# Autodesk Inventor assembly: Wrist
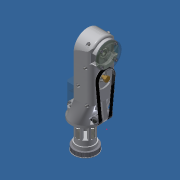
[picture p0: Inventor's stored thumbnail of the model, 180x180]
Saved by Autodesk Inventor 2016 (Build 200138000, 138)
## iProperties
Created: 2015-08-25
Part Number: Wrist
Material: Generisch
Document SubType Name: Assembly
Designer: 4ndreas
Mass: 901.602 g
Surface Area: 1453.73 cm^2
Volume: 401.24 cm^3
Density: 2.24704 g/cm^3
Author: 4ndreas
## Documents named in this file (29)
- C:\Users\4ndreas\Documents\Inventor\RobotARM v2\v4\Wrist.iam
- C:\Users\4ndreas\Documents\Inventor\RobotARM v2\v4\Wrist_A.ipt
- C:\Users\4ndreas\Documents\Inventor\RobotARM v2\v4\Nema17 48.ipt
- C:\Users\4ndreas\Documents\Inventor\RobotARM v2\v4\Wrist\Konstruktions-Assistent\Übertragung des Zahnriemens1.iam
- C:\Users\4ndreas\Documents\Inventor\RobotARM v2\v4\DIN 625 SKF - SKF 624_flansch.ipt
- C:\Users\4ndreas\Documents\Inventor\RobotARM v2\v4\Synchrone Riemenscheibe16.ipt
- C:\Users\4ndreas\Documents\Inventor\Content Center Files\R2014\de-DE\DIN BEARING(1)\DIN 625 SKF - SKF 626.ipt
- C:\Users\4ndreas\Documents\Inventor\Content Center Files\R2014\de-DE\DIN BEARING(1)\DIN 625 SKF - SKF 608.ipt
- C:\Users\4ndreas\Documents\Inventor\Content Center Files\R2014\de-DE\DIN BEARING(1)\DIN 625 SKF - SKF 624.ipt
- C:\Users\4ndreas\Documents\Inventor\Content Center Files\R2014\de-DE\ISO 7380-1\ISO 7380-1 - M4 x 30.ipt
- C:\Users\4ndreas\Documents\Inventor\Content Center Files\R2014\de-DE\ISO 7380-1\ISO 7380-1 - M4 x 35.ipt
- C:\Users\4ndreas\Documents\Inventor\RobotARM v2\v4\Twisted_Belt.ipt
- C:\Users\4ndreas\Documents\Inventor\RobotARM v2\v2\encoder.iam
- C:\Users\4ndreas\Documents\Inventor\Content Center Files\R2014\de-DE\DIN 125-1  A\DIN 125 - A 4,3.ipt
- C:\Users\4ndreas\Documents\Inventor\Content Center Files\R2014\de-DE\DIN 912\DIN 912 - M4 x 0,7 x 20 x 18,25.ipt
- C:\Users\4ndreas\Documents\Inventor\Content Center Files\R2014\de-DE\DIN 934\DIN 934 - M4 x 0,7.ipt
- C:\Users\4ndreas\Documents\Inventor\Content Center Files\R2014\de-DE\DIN 912\DIN 912 - M3 x 0,5 x 16 x 14,75.ipt
- C:\Users\4ndreas\Documents\Inventor\Content Center Files\R2014\de-DE\DIN 125-1  A\DIN 125 - A 3,2.ipt
- C:\Users\4ndreas\Documents\Inventor\Content Center Files\R2014\de-DE\DIN 7991(2)\DIN 7991 - M3x10.ipt
- C:\Users\4ndreas\Documents\Inventor\Content Center Files\R2014\de-DE\DIN 912\DIN 912 - M4 x 0,7 x 40 x 20.ipt
- C:\Users\4ndreas\Documents\Inventor\RobotARM v2\v4\RotoatorGear.ipt
- C:\Users\4ndreas\Documents\Inventor\Content Center Files\R2014\de-DE\DIN 933\DIN 933 - M4  x 30.ipt
- C:\Users\4ndreas\Documents\Inventor\Content Center Files\R2014\de-DE\DIN 912\DIN 912 - M4 x 0,7 x 30 x 20.ipt
- C:\Users\4ndreas\Documents\Inventor\RobotARM v2\v4\T25-06-44_2.ipt
- C:\Users\4ndreas\Documents\Inventor\RobotARM v2\v4\Bolzen6mm.ipt
- C:\Users\4ndreas\Documents\Inventor\RobotARM v2\Diszanzbolzen_M4x20.ipt
- C:\Users\4ndreas\Documents\Inventor\RobotARM v2\v4\DIN 912 - M4 x 0,7 x55.ipt
- C:\Users\4ndreas\Documents\Inventor\Content Center Files\R2014\de-DE\DIN 985\DIN 985 - M4.ipt
- C:\Users\4ndreas\Documents\Inventor\Content Center Files\R2014\de-DE\DIN 562\DIN 562 - M4 x 7.ipt
## Components (68 placed, 28 different names)
1. Wrist_A:1 — Passend:1, Winkel:1, Passend:2, Winkel:2, Fluchtend:1, Fluchtend:2, Passend:5, Passend:8, Passend:11, Passend:12, Passend:14, Passend:15, Fluchtend:4, Passend:20, Passend:22, Passend:23, Passend:24, Passend:34, Passend:39, Passend:40, Winkel:3, Passend:51, Passend:54, Passend:58, Passend:59, Passend:61, Passend:62, Passend:66, Passend:67, Passend:70, Passend:71, Passend:77, Passend:78, Passend:79, Passend:80, Passend:81, Passend:82, Passend:83, Passend:84, Passend:85, Passend:94, Passend:95, Passend:96, Passend:97, Passend:102, Passend:103, Passend:105, Passend:120, Passend:121, Passend:122, Passend:123, Passend:124, Passend:125, Passend:126, Passend:127, Passend:128, Passend:129, Passend:130, Passend:131, Passend:159, Passend:161, Passend:162
2. Nema17 48:1 — Passend:1, Winkel:1, Fluchtend:1, Passend:6, Passend:7, Passend:98, Passend:99, Passend:100, Passend:101
3. Übertragung des Zahnriemens:1 [sub-assembly] — Passend:13, Passend:21, Passend:27, Passend:31, Passend:48
4. F624 ZZ 4x13x5:2 — Passend:3, Passend:4, Passend:35
5. F624 ZZ 4x13x5:3 — Passend:3, Passend:4, Passend:5, Passend:8, Fluchtend:6, Passend:36
6. Synchrone Riemenscheibe1:1 — Passend:6, Passend:7, Fluchtend:5, Fluchtend:8, Passend:38
7. F624 ZZ 4x13x5:4 — Passend:9, Passend:10, Passend:11, Passend:12
8. F624 ZZ 4x13x5:5 — Passend:9, Passend:10, Passend:44
9. Synchrone Riemenscheibe1:2 — Passend:13, Passend:19
10. DIN 625 SKF SKF 626:1 — Passend:14, Fluchtend:4, Passend:154, Passend:157
11. DIN 625 SKF SKF 626:2 — Passend:15, Passend:19, Passend:20
12. DIN 625 SKF SKF 608:1 — Passend:22, Passend:24
13. DIN 625 SKF SKF 608:2 — Passend:21, Passend:23
14. DIN 625 SKF SKF 624:6 — Passend:25, Passend:26, Passend:27, Passend:32
15. DIN 625 SKF SKF 624:7 — Passend:25, Passend:26
16. DIN 125-1 A A 4,3:6
17. ISO 7380-1 M4 x 30:1 — Passend:31, Passend:32, Passend:160
18. ISO 7380-1 M4 x 35:1 — Passend:34, Passend:35, Passend:43
19. Twisted_Belt:1 — Fluchtend:5, Fluchtend:6, Passend:36, Fluchtend:8, Passend:38
20. DIN 985 - ersetzt durch DIN EN ISO 10511 M4:1 — Passend:43, Passend:44
21. encoder:1 [sub-assembly] — Passend:48, Winkel:3, Winkel:4, Passend:104, Passend:159
22. DIN 912 - ersetzt durch DIN EN ISO 4762 M4 x 55:1 — Passend:51, Passend:52, Passend:53, Passend:75
23. DIN 912 - ersetzt durch DIN EN ISO 4762 M4 x 55:2 — Passend:56, Passend:59, Passend:64, Passend:73
24. DIN 912 - ersetzt durch DIN EN ISO 4762 M4 x 55:3 — Passend:57, Passend:58, Passend:65, Passend:74
25. DIN 125-1 A A 4,3:1 — Passend:52, Passend:53, Passend:54
26. DIN 125-1 A A 4,3:2 — Passend:57, Passend:65, Passend:66
27. DIN 125-1 A A 4,3:3 — Passend:56, Passend:64, Passend:67
28. DIN 125-1 A A 4,3:4 — Passend:60, Passend:62, Passend:63
29. DIN 912 - ersetzt durch DIN EN ISO 4762 M4 x 40:5 — Passend:60, Passend:61, Passend:63, Passend:72
30. DIN 912 - ersetzt durch DIN EN ISO 4762 M4 x 20:1 — Passend:68, Passend:69, Passend:71, Passend:76
31. DIN 125-1 A A 4,3:5 — Passend:68, Passend:69, Passend:70
32. DIN 934 - ersetzt durch DIN EN 24032/28673/28674 M4:1 — Passend:72, Passend:79, Passend:85
33. DIN 934 - ersetzt durch DIN EN 24032/28673/28674 M4:2 — Passend:73, Passend:80, Passend:84
34. DIN 934 - ersetzt durch DIN EN 24032/28673/28674 M4:3 — Passend:74, Passend:81, Passend:82
35. DIN 934 - ersetzt durch DIN EN 24032/28673/28674 M4:4 — Passend:75, Passend:83
36. DIN 934 - ersetzt durch DIN EN 24032/28673/28674 M4:5 — Passend:76, Passend:77, Passend:78
37. DIN 912 - ersetzt durch DIN EN ISO 4762 M3 x 16:1 — Passend:89, Passend:90, Passend:101
38. DIN 912 - ersetzt durch DIN EN ISO 4762 M3 x 16:2 — Passend:88, Passend:91, Passend:99
39. DIN 912 - ersetzt durch DIN EN ISO 4762 M3 x 16:3 — Passend:87, Passend:92, Passend:98
40. DIN 912 - ersetzt durch DIN EN ISO 4762 M3 x 16:4 — Passend:86, Passend:93, Passend:100
41. DIN 125-1 A A 3,2:1 — Passend:86, Passend:93, Passend:94
42. DIN 125-1 A A 3,2:2 — Passend:89, Passend:90, Passend:97
43. DIN 125-1 A A 3,2:3 — Passend:88, Passend:91, Passend:96
44. DIN 125-1 A A 3,2:4 — Passend:87, Passend:92, Passend:95
45. DIN 7991 M3x10:1 — Passend:105, Fluchtend:11, Fluchtend:12
46. DIN 7991 M3x10:2 — Passend:103, Fluchtend:10, Fluchtend:11
47. DIN 7991 M3x10:3 — Passend:104, Fluchtend:12
48. DIN 7991 M3x10:4 — Passend:102, Fluchtend:10
49. RotoatorGear:1 — Passend:120, Passend:121, Passend:122, Passend:136, Passend:137, Passend:138, Passend:139, Passend:148, Passend:149
50. DIN 933 - ersetzt durch DIN EN 24017 M4  x 30:4 — Passend:123, Fluchtend:16, Fluchtend:17, Passend:130, Passend:131, Passend:135
51. DIN 933 - ersetzt durch DIN EN 24017 M4  x 30:3 — Passend:124, Fluchtend:17, Passend:129, Passend:134
52. DIN 933 - ersetzt durch DIN EN 24017 M4  x 30:2 — Passend:125, Fluchtend:15, Passend:128, Passend:133
53. DIN 933 - ersetzt durch DIN EN 24017 M4  x 30:1 — Passend:126, Fluchtend:15, Fluchtend:16, Passend:127, Passend:132
54. Diszanzbolzen_M4x20:5 — Passend:132, Passend:138, Passend:152
55. Diszanzbolzen_M4x20:6 — Passend:133, Passend:139, Passend:151
56. Diszanzbolzen_M4x20:7 — Passend:134, Passend:137, Passend:150
57. Diszanzbolzen_M4x20:8 — Passend:135, Passend:136
58. DIN 125-1 A A 4,3:7
59. DIN 125-1 A A 4,3:8
60. DIN 125-1 A A 4,3:9
61. DIN 125-1 A A 4,3:10
62. DIN 912 - ersetzt durch DIN EN ISO 4762 M4 x 30:1 — Fluchtend:20, Passend:150
63. DIN 912 - ersetzt durch DIN EN ISO 4762 M4 x 30:2 — Fluchtend:19, Fluchtend:20, Passend:152
64. DIN 912 - ersetzt durch DIN EN ISO 4762 M4 x 30:3 — Fluchtend:18, Fluchtend:19, Passend:151
65. DIN 912 - ersetzt durch DIN EN ISO 4762 M4 x 30:4 — Passend:148, Passend:149, Fluchtend:18
66. T25-06-44_2:1 — Passend:154, Passend:155, Passend:156, Passend:158
67. Bolzen6mm:1 — Passend:155, Passend:156, Passend:157, Passend:158
68. DIN 562 M4:1 — Passend:160, Passend:161, Passend:162
## Relationships (155: Mate 136, Flush 15, Angle 4)
- Passend:1 [Mate]: Wrist_A:1 ↔ Nema17 48:1
- Winkel:1 [Angle] (0 deg): Wrist_A:1 ↔ Nema17 48:1
- Passend:2 [Mate]: Wrist_A:1
- Winkel:2 [Angle] (90 deg): Wrist_A:1
- Fluchtend:1 [Flush] (20 mm): Wrist_A:1 ↔ Nema17 48:1
- Fluchtend:2 [Flush]: Wrist_A:1
- Passend:3 [Mate]: F624 ZZ 4x13x5:2 ↔ F624 ZZ 4x13x5:3
- Passend:4 [Mate]: F624 ZZ 4x13x5:2 ↔ F624 ZZ 4x13x5:3
- Passend:5 [Mate]: Wrist_A:1 ↔ F624 ZZ 4x13x5:3
- Passend:6 [Mate] (4.5 mm): Nema17 48:1 ↔ Synchrone Riemenscheibe1:1
- Passend:7 [Mate]: Nema17 48:1 ↔ Synchrone Riemenscheibe1:1
- Passend:8 [Mate]: Wrist_A:1 ↔ F624 ZZ 4x13x5:3
- Passend:9 [Mate]: F624 ZZ 4x13x5:4 ↔ F624 ZZ 4x13x5:5
- Passend:10 [Mate]: F624 ZZ 4x13x5:4 ↔ F624 ZZ 4x13x5:5
- Passend:11 [Mate]: Wrist_A:1 ↔ F624 ZZ 4x13x5:4
- Passend:12 [Mate]: Wrist_A:1 ↔ F624 ZZ 4x13x5:4
- Passend:13 [Mate]: Übertragung des Zahnriemens:1 ↔ Synchrone Riemenscheibe1:2
- Passend:14 [Mate]: Wrist_A:1 ↔ DIN 625 SKF SKF 626:1
- Passend:15 [Mate]: Wrist_A:1 ↔ DIN 625 SKF SKF 626:2
- Fluchtend:4 [Flush]: Wrist_A:1 ↔ DIN 625 SKF SKF 626:1
- Passend:19 [Mate]: Synchrone Riemenscheibe1:2 ↔ DIN 625 SKF SKF 626:2
- Passend:20 [Mate]: Wrist_A:1 ↔ DIN 625 SKF SKF 626:2
- Passend:21 [Mate]: Übertragung des Zahnriemens:1 ↔ DIN 625 SKF SKF 608:2
- Passend:22 [Mate]: Wrist_A:1 ↔ DIN 625 SKF SKF 608:1
- Passend:23 [Mate]: Wrist_A:1 ↔ DIN 625 SKF SKF 608:2
- Passend:24 [Mate]: Wrist_A:1 ↔ DIN 625 SKF SKF 608:1
- Passend:25 [Mate]: DIN 625 SKF SKF 624:6 ↔ DIN 625 SKF SKF 624:7
- Passend:26 [Mate]: DIN 625 SKF SKF 624:6 ↔ DIN 625 SKF SKF 624:7
- Passend:27 [Mate]: Übertragung des Zahnriemens:1 ↔ DIN 625 SKF SKF 624:6
- [Mate]: Übertragung des Zahnriemens:1 ↔ DIN 125-1 A A 4,3:6
- [Mate]: DIN 625 SKF SKF 624:7 ↔ DIN 125-1 A A 4,3:6
- Passend:31 [Mate]: Übertragung des Zahnriemens:1 ↔ ISO 7380-1 M4 x 30:1
- Passend:32 [Mate]: DIN 625 SKF SKF 624:6 ↔ ISO 7380-1 M4 x 30:1
- [Mate]: Wrist_A:1 ↔ DIN 125-1 A A 4,3:6
- Passend:34 [Mate]: Wrist_A:1 ↔ ISO 7380-1 M4 x 35:1
- Passend:35 [Mate]: F624 ZZ 4x13x5:2 ↔ ISO 7380-1 M4 x 35:1
- Fluchtend:5 [Flush] (3.5 mm): Synchrone Riemenscheibe1:1 ↔ Twisted_Belt:1
- Fluchtend:6 [Flush] (-5 mm): F624 ZZ 4x13x5:3 ↔ Twisted_Belt:1
- Passend:36 [Mate]: F624 ZZ 4x13x5:3 ↔ Twisted_Belt:1
- Fluchtend:8 [Flush]: Synchrone Riemenscheibe1:1 ↔ Twisted_Belt:1
- Passend:38 [Mate]: Synchrone Riemenscheibe1:1 ↔ Twisted_Belt:1
- Passend:39 [Mate]: Wrist_A:1
- Passend:40 [Mate]: Wrist_A:1
- Passend:41 [Mate]
- Passend:42 [Mate]
- Passend:43 [Mate]: ISO 7380-1 M4 x 35:1 ↔ DIN 985 - ersetzt durch DIN EN ISO 10511 M4:1
- Passend:44 [Mate]: F624 ZZ 4x13x5:5 ↔ DIN 985 - ersetzt durch DIN EN ISO 10511 M4:1
- Passend:48 [Mate]: Übertragung des Zahnriemens:1 ↔ encoder:1
- Winkel:3 [Angle] (90 deg): Wrist_A:1 ↔ encoder:1
- Winkel:4 [Angle] (90 deg): encoder:1
- Passend:51 [Mate]: Wrist_A:1 ↔ DIN 912 - ersetzt durch DIN EN ISO 4762 M4 x 55:1
- Passend:52 [Mate]: DIN 912 - ersetzt durch DIN EN ISO 4762 M4 x 55:1 ↔ DIN 125-1 A A 4,3:1
- Passend:53 [Mate]: DIN 912 - ersetzt durch DIN EN ISO 4762 M4 x 55:1 ↔ DIN 125-1 A A 4,3:1
- Passend:54 [Mate]: Wrist_A:1 ↔ DIN 125-1 A A 4,3:1
- Passend:56 [Mate]: DIN 912 - ersetzt durch DIN EN ISO 4762 M4 x 55:2 ↔ DIN 125-1 A A 4,3:3
- Passend:57 [Mate]: DIN 912 - ersetzt durch DIN EN ISO 4762 M4 x 55:3 ↔ DIN 125-1 A A 4,3:2
- Passend:58 [Mate]: Wrist_A:1 ↔ DIN 912 - ersetzt durch DIN EN ISO 4762 M4 x 55:3
- Passend:59 [Mate]: Wrist_A:1 ↔ DIN 912 - ersetzt durch DIN EN ISO 4762 M4 x 55:2
- Passend:60 [Mate]: DIN 125-1 A A 4,3:4 ↔ DIN 912 - ersetzt durch DIN EN ISO 4762 M4 x 40:5
- Passend:61 [Mate]: Wrist_A:1 ↔ DIN 912 - ersetzt durch DIN EN ISO 4762 M4 x 40:5
- Passend:62 [Mate]: Wrist_A:1 ↔ DIN 125-1 A A 4,3:4
- Passend:63 [Mate]: DIN 125-1 A A 4,3:4 ↔ DIN 912 - ersetzt durch DIN EN ISO 4762 M4 x 40:5
- Passend:64 [Mate]: DIN 912 - ersetzt durch DIN EN ISO 4762 M4 x 55:2 ↔ DIN 125-1 A A 4,3:3
- Passend:65 [Mate]: DIN 912 - ersetzt durch DIN EN ISO 4762 M4 x 55:3 ↔ DIN 125-1 A A 4,3:2
- Passend:66 [Mate]: Wrist_A:1 ↔ DIN 125-1 A A 4,3:2
- Passend:67 [Mate]: Wrist_A:1 ↔ DIN 125-1 A A 4,3:3
- Passend:68 [Mate]: DIN 912 - ersetzt durch DIN EN ISO 4762 M4 x 20:1 ↔ DIN 125-1 A A 4,3:5
- Passend:69 [Mate]: DIN 912 - ersetzt durch DIN EN ISO 4762 M4 x 20:1 ↔ DIN 125-1 A A 4,3:5
- Passend:70 [Mate]: Wrist_A:1 ↔ DIN 125-1 A A 4,3:5
- Passend:71 [Mate]: Wrist_A:1 ↔ DIN 912 - ersetzt durch DIN EN ISO 4762 M4 x 20:1
- Passend:72 [Mate]: DIN 912 - ersetzt durch DIN EN ISO 4762 M4 x 40:5 ↔ DIN 934 - ersetzt durch DIN EN 24032/28673/28674 M4:1
- Passend:73 [Mate]: DIN 912 - ersetzt durch DIN EN ISO 4762 M4 x 55:2 ↔ DIN 934 - ersetzt durch DIN EN 24032/28673/28674 M4:2
- Passend:74 [Mate]: DIN 912 - ersetzt durch DIN EN ISO 4762 M4 x 55:3 ↔ DIN 934 - ersetzt durch DIN EN 24032/28673/28674 M4:3
- Passend:75 [Mate]: DIN 912 - ersetzt durch DIN EN ISO 4762 M4 x 55:1 ↔ DIN 934 - ersetzt durch DIN EN 24032/28673/28674 M4:4
- Passend:76 [Mate]: DIN 912 - ersetzt durch DIN EN ISO 4762 M4 x 20:1 ↔ DIN 934 - ersetzt durch DIN EN 24032/28673/28674 M4:5
- Passend:77 [Mate]: Wrist_A:1 ↔ DIN 934 - ersetzt durch DIN EN 24032/28673/28674 M4:5
- Passend:78 [Mate]: Wrist_A:1 ↔ DIN 934 - ersetzt durch DIN EN 24032/28673/28674 M4:5
- Passend:79 [Mate]: Wrist_A:1 ↔ DIN 934 - ersetzt durch DIN EN 24032/28673/28674 M4:1
- Passend:80 [Mate]: Wrist_A:1 ↔ DIN 934 - ersetzt durch DIN EN 24032/28673/28674 M4:2
- Passend:81 [Mate]: Wrist_A:1 ↔ DIN 934 - ersetzt durch DIN EN 24032/28673/28674 M4:3
- Passend:82 [Mate]: Wrist_A:1 ↔ DIN 934 - ersetzt durch DIN EN 24032/28673/28674 M4:3
- Passend:83 [Mate]: Wrist_A:1 ↔ DIN 934 - ersetzt durch DIN EN 24032/28673/28674 M4:4
- Passend:84 [Mate]: Wrist_A:1 ↔ DIN 934 - ersetzt durch DIN EN 24032/28673/28674 M4:2
- Passend:85 [Mate]: Wrist_A:1 ↔ DIN 934 - ersetzt durch DIN EN 24032/28673/28674 M4:1
- Passend:86 [Mate]: DIN 912 - ersetzt durch DIN EN ISO 4762 M3 x 16:4 ↔ DIN 125-1 A A 3,2:1
- Passend:87 [Mate]: DIN 912 - ersetzt durch DIN EN ISO 4762 M3 x 16:3 ↔ DIN 125-1 A A 3,2:4
- Passend:88 [Mate]: DIN 912 - ersetzt durch DIN EN ISO 4762 M3 x 16:2 ↔ DIN 125-1 A A 3,2:3
- Passend:89 [Mate]: DIN 912 - ersetzt durch DIN EN ISO 4762 M3 x 16:1 ↔ DIN 125-1 A A 3,2:2
- Passend:90 [Mate]: DIN 912 - ersetzt durch DIN EN ISO 4762 M3 x 16:1 ↔ DIN 125-1 A A 3,2:2
- Passend:91 [Mate]: DIN 912 - ersetzt durch DIN EN ISO 4762 M3 x 16:2 ↔ DIN 125-1 A A 3,2:3
- Passend:92 [Mate]: DIN 912 - ersetzt durch DIN EN ISO 4762 M3 x 16:3 ↔ DIN 125-1 A A 3,2:4
- Passend:93 [Mate]: DIN 912 - ersetzt durch DIN EN ISO 4762 M3 x 16:4 ↔ DIN 125-1 A A 3,2:1
- Passend:94 [Mate]: Wrist_A:1 ↔ DIN 125-1 A A 3,2:1
- Passend:95 [Mate]: Wrist_A:1 ↔ DIN 125-1 A A 3,2:4
- Passend:96 [Mate]: Wrist_A:1 ↔ DIN 125-1 A A 3,2:3
- Passend:97 [Mate]: Wrist_A:1 ↔ DIN 125-1 A A 3,2:2
- Passend:98 [Mate]: Nema17 48:1 ↔ DIN 912 - ersetzt durch DIN EN ISO 4762 M3 x 16:3
- Passend:99 [Mate]: Nema17 48:1 ↔ DIN 912 - ersetzt durch DIN EN ISO 4762 M3 x 16:2
- Passend:100 [Mate]: Nema17 48:1 ↔ DIN 912 - ersetzt durch DIN EN ISO 4762 M3 x 16:4
- Passend:101 [Mate]: Nema17 48:1 ↔ DIN 912 - ersetzt durch DIN EN ISO 4762 M3 x 16:1
- Passend:102 [Mate]: Wrist_A:1 ↔ DIN 7991 M3x10:4
- Passend:103 [Mate]: Wrist_A:1 ↔ DIN 7991 M3x10:2
- Passend:104 [Mate]: encoder:1 ↔ DIN 7991 M3x10:3
- Passend:105 [Mate]: Wrist_A:1 ↔ DIN 7991 M3x10:1
- Fluchtend:10 [Flush]: DIN 7991 M3x10:2 ↔ DIN 7991 M3x10:4
- Fluchtend:11 [Flush]: DIN 7991 M3x10:1 ↔ DIN 7991 M3x10:2
- Fluchtend:12 [Flush]: DIN 7991 M3x10:1 ↔ DIN 7991 M3x10:3
- Passend:120 [Mate]: Wrist_A:1 ↔ RotoatorGear:1
- Passend:121 [Mate]: Wrist_A:1 ↔ RotoatorGear:1
- Passend:122 [Mate]: Wrist_A:1 ↔ RotoatorGear:1
- Passend:123 [Mate]: Wrist_A:1 ↔ DIN 933 - ersetzt durch DIN EN 24017 M4  x 30:4
- Passend:124 [Mate]: Wrist_A:1 ↔ DIN 933 - ersetzt durch DIN EN 24017 M4  x 30:3
- Passend:125 [Mate]: Wrist_A:1 ↔ DIN 933 - ersetzt durch DIN EN 24017 M4  x 30:2
- Passend:126 [Mate]: Wrist_A:1 ↔ DIN 933 - ersetzt durch DIN EN 24017 M4  x 30:1
- Fluchtend:15 [Flush]: DIN 933 - ersetzt durch DIN EN 24017 M4  x 30:2 ↔ DIN 933 - ersetzt durch DIN EN 24017 M4  x 30:1
- Fluchtend:16 [Flush]: DIN 933 - ersetzt durch DIN EN 24017 M4  x 30:4 ↔ DIN 933 - ersetzt durch DIN EN 24017 M4  x 30:1
- Fluchtend:17 [Flush]: DIN 933 - ersetzt durch DIN EN 24017 M4  x 30:4 ↔ DIN 933 - ersetzt durch DIN EN 24017 M4  x 30:3
- Passend:127 [Mate]: Wrist_A:1 ↔ DIN 933 - ersetzt durch DIN EN 24017 M4  x 30:1
- Passend:128 [Mate]: Wrist_A:1 ↔ DIN 933 - ersetzt durch DIN EN 24017 M4  x 30:2
- Passend:129 [Mate]: Wrist_A:1 ↔ DIN 933 - ersetzt durch DIN EN 24017 M4  x 30:3
- Passend:130 [Mate]: Wrist_A:1 ↔ DIN 933 - ersetzt durch DIN EN 24017 M4  x 30:4
- Passend:131 [Mate]: Wrist_A:1 ↔ DIN 933 - ersetzt durch DIN EN 24017 M4  x 30:4
- Passend:132 [Mate]: DIN 933 - ersetzt durch DIN EN 24017 M4  x 30:1 ↔ Diszanzbolzen_M4x20:5
- Passend:133 [Mate]: DIN 933 - ersetzt durch DIN EN 24017 M4  x 30:2 ↔ Diszanzbolzen_M4x20:6
- Passend:134 [Mate]: DIN 933 - ersetzt durch DIN EN 24017 M4  x 30:3 ↔ Diszanzbolzen_M4x20:7
- Passend:135 [Mate]: DIN 933 - ersetzt durch DIN EN 24017 M4  x 30:4 ↔ Diszanzbolzen_M4x20:8
- Passend:136 [Mate]: RotoatorGear:1 ↔ Diszanzbolzen_M4x20:8
- Passend:137 [Mate]: RotoatorGear:1 ↔ Diszanzbolzen_M4x20:7
- Passend:138 [Mate]: RotoatorGear:1 ↔ Diszanzbolzen_M4x20:5
- Passend:139 [Mate]: RotoatorGear:1 ↔ Diszanzbolzen_M4x20:6
- [Mate]: Wrist_A:1 ↔ DIN 125-1 A A 4,3:8
- [Mate]: Wrist_A:1 ↔ DIN 125-1 A A 4,3:9
- [Mate]: Wrist_A:1 ↔ DIN 125-1 A A 4,3:10
- [Mate]: Wrist_A:1 ↔ DIN 125-1 A A 4,3:7
- [Mate]: DIN 933 - ersetzt durch DIN EN 24017 M4  x 30:4 ↔ DIN 125-1 A A 4,3:7
- [Mate]: DIN 933 - ersetzt durch DIN EN 24017 M4  x 30:3 ↔ DIN 125-1 A A 4,3:8
- [Mate]: DIN 933 - ersetzt durch DIN EN 24017 M4  x 30:2 ↔ DIN 125-1 A A 4,3:9
- [Mate]: DIN 933 - ersetzt durch DIN EN 24017 M4  x 30:1 ↔ DIN 125-1 A A 4,3:10
- Passend:148 [Mate]: RotoatorGear:1 ↔ DIN 912 - ersetzt durch DIN EN ISO 4762 M4 x 30:4
- Passend:149 [Mate]: RotoatorGear:1 ↔ DIN 912 - ersetzt durch DIN EN ISO 4762 M4 x 30:4
- Fluchtend:18 [Flush]: DIN 912 - ersetzt durch DIN EN ISO 4762 M4 x 30:3 ↔ DIN 912 - ersetzt durch DIN EN ISO 4762 M4 x 30:4
- Fluchtend:19 [Flush]: DIN 912 - ersetzt durch DIN EN ISO 4762 M4 x 30:2 ↔ DIN 912 - ersetzt durch DIN EN ISO 4762 M4 x 30:3
- Fluchtend:20 [Flush]: DIN 912 - ersetzt durch DIN EN ISO 4762 M4 x 30:1 ↔ DIN 912 - ersetzt durch DIN EN ISO 4762 M4 x 30:2
- Passend:150 [Mate]: Diszanzbolzen_M4x20:7 ↔ DIN 912 - ersetzt durch DIN EN ISO 4762 M4 x 30:1
- Passend:151 [Mate]: Diszanzbolzen_M4x20:6 ↔ DIN 912 - ersetzt durch DIN EN ISO 4762 M4 x 30:3
- Passend:152 [Mate]: Diszanzbolzen_M4x20:5 ↔ DIN 912 - ersetzt durch DIN EN ISO 4762 M4 x 30:2
- Passend:154 [Mate]: DIN 625 SKF SKF 626:1 ↔ T25-06-44_2:1
- Passend:155 [Mate]: T25-06-44_2:1 ↔ Bolzen6mm:1
- Passend:156 [Mate]: T25-06-44_2:1 ↔ Bolzen6mm:1
- Passend:157 [Mate]: DIN 625 SKF SKF 626:1 ↔ Bolzen6mm:1
- Passend:158 [Mate]: T25-06-44_2:1 ↔ Bolzen6mm:1
- Passend:159 [Mate]: Wrist_A:1 ↔ encoder:1
- Passend:160 [Mate]: ISO 7380-1 M4 x 30:1 ↔ DIN 562 M4:1
- Passend:161 [Mate]: Wrist_A:1 ↔ DIN 562 M4:1
- Passend:162 [Mate]: Wrist_A:1 ↔ DIN 562 M4:1
